# Autodesk Inventor assembly: 111-01
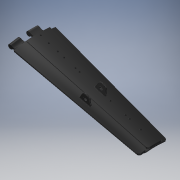
[picture p0: Inventor's stored thumbnail of the model, 180x180]
Saved by Autodesk Inventor 2019 (Build 230136000, 136)
## iProperties
Created: 2017-03-16
Part Number: 111-01
Document SubType Name: Assembly
Designer: wangru
Mass: 159.679 g
Surface Area: 259.251 cm^2
Volume: 18.1041 cm^3
Density: 8.82006 g/cm^3
Author: wangru
## Documents named in this file (5)
- C:\Samples\Jet Engine Model\Workspace\Blade.iam
- C:\Samples\Jet Engine Model\Workspace\Blade-1.ipt
- C:\Samples\Jet Engine Model\Workspace\Blade-2.ipt
- C:\Samples\Jet Engine Model\Workspace\Blade-3.ipt
- C:\Users\t_crawk\Documents\Inventor\Sample Files\Jet Engine\CC\Rivet GB_T 1014-1986-2 X 4.ipt
## Components (8 placed, 4 different names)
1. Blade-2:1 — Mate:1
2. Blade-3:1 — Mate:5, Mate:7, Mate:8, Mate:9, Mate:10, Mate:11, Mate:12
3. Blade-1:1 — Mate:1
4. Rivet GB/T 1014-1986 2 X 4:1 — Mate:8
5. Rivet GB/T 1014-1986 2 X 4:2 — Mate:12
6. Rivet GB/T 1014-1986 2 X 4:3 — Mate:11
7. Rivet GB/T 1014-1986 2 X 4:4 — Mate:10
8. Rivet GB/T 1014-1986 2 X 4:5 — Mate:9
## Relationships (9: Mate 8, Flush 1)
- Mate:1: Blade-2:1 ↔ Blade-1:1
- Mate:5: Blade-3:1
- Mate:7: Blade-3:1
- Flush:1 (-6.75 mm)
- Mate:8: Blade-3:1 ↔ Rivet GB/T 1014-1986 2 X 4:1
- Mate:9: Blade-3:1 ↔ Rivet GB/T 1014-1986 2 X 4:5
- Mate:10: Blade-3:1 ↔ Rivet GB/T 1014-1986 2 X 4:4
- Mate:11: Blade-3:1 ↔ Rivet GB/T 1014-1986 2 X 4:3
- Mate:12: Blade-3:1 ↔ Rivet GB/T 1014-1986 2 X 4:2
